# Autodesk Inventor assembly: Nema17MetGearbox
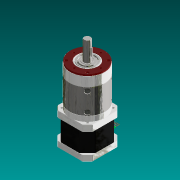
[picture p0: Inventor's stored thumbnail of the model, 180x180]
Saved by Autodesk Inventor 2020.3 (Build 243373000, 373)
## iProperties
Created: 2020-05-14
Part Number: Nema17MetGearbox
Document SubType Name: Assembly
Designer: Svend
Author: Svend
## Documents named in this file (4)
- C:\Users\Svend\OneDrive\Documents\GitHub\BeerMinder\3D-model\subAssembly\Nema17MetGearbox.iam
- C:\Users\Svend\OneDrive\Documents\GitHub\BeerMinder\3D-model\stepper motors\42BYG Stepper Motor.ipt
- C:\Users\Svend\OneDrive\Documents\GitHub\BeerMinder\3D-model\gearbox\gearbox.iam
- C:\Users\Svend\OneDrive\Documents\GitHub\BeerMinder\3D-model\Base (Axis 1)\gearboxspacer.ipt
## Components (3 placed, 3 different names)
1. 42BYG Stepper Motor:1 — Mate:1, Mate:2, Angle:1
2. gearbox:1 [sub-assembly] — Mate:1, Mate:2, Angle:1, Flush:1, Flush:2, Mate:3, Mate:4
3. gearboxspacer:1 — Flush:1, Flush:2, Mate:3, Mate:4
## Relationships (7: Mate 4, Flush 2, Angle 1)
- Mate:1: 42BYG Stepper Motor:1 ↔ gearbox:1
- Mate:2: 42BYG Stepper Motor:1 ↔ gearbox:1
- Angle:1 (45 deg): 42BYG Stepper Motor:1 ↔ gearbox:1
- Flush:1: gearbox:1 ↔ gearboxspacer:1
- Flush:2: gearbox:1 ↔ gearboxspacer:1
- Mate:3: gearbox:1 ↔ gearboxspacer:1
- Mate:4: gearbox:1 ↔ gearboxspacer:1
